# Autodesk Inventor assembly: 4 Omni Wheel
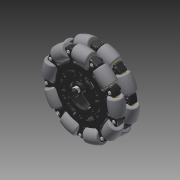
[picture p0: Inventor's stored thumbnail of the model, 180x180]
Saved by Autodesk Inventor 2015 SP1 (Build 190203100, 203)
## iProperties
Created: 2013-01-03
Part Number: 4 Omni Wheel
Document SubType Name: Assembly
Designer: Nemo
Author: Nemo
## Documents named in this file (6)
- C:\Users\datenney\Documents\GitHub\CAD\COTSParts\Wheels\VexPro Omni Wheels\4 Omni Wheel.iam
- C:\Users\datenney\Documents\GitHub\CAD\COTSParts\Wheels\VexPro Omni Wheels\Components\Omni Wheel Inside 4 in.ipt
- C:\Users\datenney\Documents\GitHub\CAD\COTSParts\Wheels\VexPro Omni Wheels\Components\Omni Wheel Outside 4 in.ipt
- C:\Users\datenney\Documents\GitHub\CAD\COTSParts\Fasteners\Hex Standoff 8-32 x750.ipt
- C:\Users\datenney\Documents\GitHub\CAD\COTSParts\Wheels\VexPro Omni Wheels\Components\Omni Roller 4 in.iam
- C:\Users\datenney\Documents\GitHub\CAD\COTSParts\Wheels\VexPro Omni Wheels\Components\Omni Wheel Screw for VexPro.ipt
## Components (45 placed, 5 different names)
1. Omni Wheel Inside 4 in:1 — Mate:1, Mate:2, Flush:1, Flush:2, Mate:3, Mate:4, Mate:5, Mate:8
2. Omni Wheel Outside 4 in:1 — Mate:1, Flush:1, Mate:4, Mate:6, Insert:2
3. Omni Wheel Outside 4 in:2 — Mate:2, Flush:2, Mate:3, Angle:1, Insert:1, Mate:7, Insert:3
4. Hex Standoff 8-32 x750:1 — Angle:1, Insert:1
5. Hex Standoff 8-32 x750:2
6. Hex Standoff 8-32 x750:3
7. Hex Standoff 8-32 x750:4
8. Hex Standoff 8-32 x750:5
9. Hex Standoff 8-32 x750:6
10. Omni Roller 4 in:2 [sub-assembly] — Mate:5, Mate:6
11. Omni Roller 4 in:3 [sub-assembly] — Mate:7, Mate:8
12. Omni Roller 4 in:4 [sub-assembly]
13. Omni Roller 4 in:5 [sub-assembly]
14. Omni Roller 4 in:6 [sub-assembly]
15. Omni Roller 4 in:7 [sub-assembly]
16. Omni Roller 4 in:8 [sub-assembly]
17. Omni Roller 4 in:9 [sub-assembly]
18. Omni Roller 4 in:10 [sub-assembly]
19. Omni Roller 4 in:11 [sub-assembly]
20. Omni Roller 4 in:12 [sub-assembly]
21. Omni Roller 4 in:13 [sub-assembly]
22. Omni Roller 4 in:14 [sub-assembly]
23. Omni Roller 4 in:15 [sub-assembly]
24. Omni Roller 4 in:16 [sub-assembly]
25. Omni Roller 4 in:17 [sub-assembly]
26. Omni Roller 4 in:18 [sub-assembly]
27. Omni Roller 4 in:19 [sub-assembly]
28. Omni Wheel Screw for VexPro:2 — Insert:3
29. Omni Wheel Screw for VexPro:1 — Insert:2
30. Omni Wheel Screw for VexPro:3
31. Omni Wheel Screw for VexPro:4
32. Omni Wheel Screw for VexPro:5
33. Omni Wheel Screw for VexPro:6
34. Omni Wheel Screw for VexPro:7
35. Omni Wheel Screw for VexPro:8
36. Omni Wheel Screw for VexPro:9
37. Omni Wheel Screw for VexPro:10
38. Omni Wheel Screw for VexPro:11
39. Omni Wheel Screw for VexPro:12
40. Omni Wheel Screw for VexPro:13
41. Omni Wheel Screw for VexPro:14
42. Omni Wheel Screw for VexPro:15
43. Omni Wheel Screw for VexPro:16
44. Omni Wheel Screw for VexPro:17
45. Omni Wheel Screw for VexPro:18
## Component patterns: (6 elements, first: Hex Standoff 8-32 x750:1), (9 elements, first: Omni Roller 4 in:2 + Omni Roller 4 in:3), (9 elements, first: Omni Wheel Screw for VexPro:2 + Omni Wheel Screw for VexPro:1)
## Relationships (14: Mate 8, Insert 3, Flush 2, Angle 1)
- Mate:1: Omni Wheel Inside 4 in:1 ↔ Omni Wheel Outside 4 in:1
- Mate:2: Omni Wheel Inside 4 in:1 ↔ Omni Wheel Outside 4 in:2
- Flush:1: Omni Wheel Inside 4 in:1 ↔ Omni Wheel Outside 4 in:1
- Flush:2: Omni Wheel Inside 4 in:1 ↔ Omni Wheel Outside 4 in:2
- Mate:3: Omni Wheel Inside 4 in:1 ↔ Omni Wheel Outside 4 in:2
- Angle:1 (0 deg): Omni Wheel Outside 4 in:2 ↔ Hex Standoff 8-32 x750:1
- Insert:1: Omni Wheel Outside 4 in:2 ↔ Hex Standoff 8-32 x750:1
- Mate:4: Omni Wheel Inside 4 in:1 ↔ Omni Wheel Outside 4 in:1
- Mate:5: Omni Wheel Inside 4 in:1 ↔ Omni Roller 4 in:2
- Mate:6 (0.1905 mm): Omni Wheel Outside 4 in:1 ↔ Omni Roller 4 in:2
- Mate:7: Omni Wheel Outside 4 in:2 ↔ Omni Roller 4 in:3
- Mate:8 (0.2032 mm): Omni Wheel Inside 4 in:1 ↔ Omni Roller 4 in:3
- Insert:2: Omni Wheel Outside 4 in:1 ↔ Omni Wheel Screw for VexPro:1
- Insert:3: Omni Wheel Outside 4 in:2 ↔ Omni Wheel Screw for VexPro:2
